# Autodesk Inventor assembly: Everything
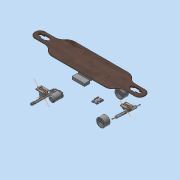
[picture p0: Inventor's stored thumbnail of the model, 180x180]
Saved by Autodesk Inventor 2017 (Build 210142000, 142)
## iProperties
Created: 2016-01-09
Part Number: Everything
Document SubType Name: Assembly
Designer: JoshuaYuan
Author: JoshuaYuan
## Documents named in this file (9)
- C:\Other Project Stuff\Longboard\Everything.iam
- C:\Other Project Stuff\Longboard\TruckAssembly.iam
- C:\Other Project Stuff\Longboard\arduino_uno.ipt
- C:\Other Project Stuff\Longboard\battery.ipt
- C:\Other Project Stuff\Longboard\Wheels.ipt
- C:\Other Project Stuff\Longboard\bearing_ABEC_7.ipt
- C:\Other Project Stuff\Longboard\50cal_truck.ipt
- C:\Other Project Stuff\Longboard\50cal_baseplate.ipt
- C:\Other Project Stuff\Longboard\Deck.ipt
## Components (16 placed, 8 different names)
1. TruckAssembly:1 [sub-assembly] — truck axle insert
2. arduino_uno:1
3. battery:1
4. battery:2
5. Wheels:1 — outer bearing insert, inner bearing insert, truck axle insert
6. Wheels:2 — Insert:5, Insert:6
7. Wheels:3 — Insert:3, Insert:4
8. bearing_ABEC_7:1 — inner bearing insert
9. bearing_ABEC_7:2 — outer bearing insert
10. bearing_ABEC_7:3 — Insert:4
11. bearing_ABEC_7:4 — Insert:5
12. bearing_ABEC_7:5 — Insert:6
13. bearing_ABEC_7:6 — Insert:3
14. 50cal_truck:1 — Mate:1, Mate:2
15. 50cal_baseplate:1 — Mate:1, Mate:2
16. Deck:1
## Relationships (9: Insert 7, Mate 2)
- outer bearing insert [Insert]: Wheels:1 ↔ bearing_ABEC_7:2
- inner bearing insert [Insert]: Wheels:1 ↔ bearing_ABEC_7:1
- Insert:3: Wheels:3 ↔ bearing_ABEC_7:6
- Insert:4: Wheels:3 ↔ bearing_ABEC_7:3
- Insert:5: Wheels:2 ↔ bearing_ABEC_7:4
- Insert:6: Wheels:2 ↔ bearing_ABEC_7:5
- Mate:1: 50cal_truck:1 ↔ 50cal_baseplate:1
- Mate:2: 50cal_truck:1 ↔ 50cal_baseplate:1
- truck axle insert [Insert] (2 mm): TruckAssembly:1 ↔ Wheels:1
